# Autodesk Inventor assembly: X_CarriageFWDBearing_V2_1_Short
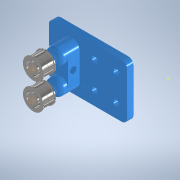
[picture p0: Inventor's stored thumbnail of the model, 180x180]
Saved by Autodesk Inventor 2022 (Build 260153000, 153)
## iProperties
Created: 2021-06-13
Part Number: X_CarriageFWDBearing_V2_1_Short
Document SubType Name: Assembly
Designer: Jorian Brusind
Author: Jorian Brusind
## Documents named in this file (6)
- C:\Users\Jorian Brusind\Documents\GitHub\HyperRail\Inventor Files\X_CarriageFWDBearing_V2_1_Short.iam
- C:\Users\Jorian Brusind\Documents\GitHub\HyperRail\Inventor Files\4mm_Roller_Spacer_simple.ipt
- C:\Users\Jorian Brusind\Documents\GitHub\HyperRail\Inventor Files\X_Carriage_Plate_Short.ipt
- C:\Users\Jorian Brusind\Documents\GitHub\HyperRail\Inventor Files\miniature-ball-bearings-metric-series-flanged-1.snapshot.1\F606ZZFlanged\F608 - 8 x 22 x 7.ipt
- C:\Users\Jorian Brusind\Documents\GitHub\PersonalProjects\HyperRail\Inventor Files\miniature-ball-bearings-metric-series-flanged-1.snapshot.1\F606ZZFlanged.ipt
- C:\Users\Jorian Brusind\Documents\GitHub\HyperRail\Inventor Files\Metric bolt\Bolt M5 45mm.ipt
## Components (8 placed, 4 different names)
1. X_Carriage_Plate_Short:1 — Mate:6, Mate:9, Angle:1, Mate:20
2. 4mm_Roller_Spacer_simple:1 — Mate:6, Mate:9, Angle:1, Mate:14, Mate:15, Mate:16, Mate:17, Mate:18, Mate:19
3. F608 - 8 x 22 x 7:4 — Mate:10, Mate:11
4. F608 - 8 x 22 x 7:5 — Mate:10, Mate:11, Mate:14, Mate:15
5. F608 - 8 x 22 x 7:6 — Mate:16
6. F608 - 8 x 22 x 7:7 — Mate:17
7. Bolt M5 45mm:1 — Mate:19, Mate:20, Flush:1
8. Bolt M5 45mm:2 — Mate:18, Flush:1
## Relationships (15: Mate 13, Angle 1, Flush 1)
- Mate:6: X_Carriage_Plate_Short:1 ↔ 4mm_Roller_Spacer_simple:1
- Mate:9 (-12.5 mm): X_Carriage_Plate_Short:1 ↔ 4mm_Roller_Spacer_simple:1
- Angle:1 (0 deg): X_Carriage_Plate_Short:1 ↔ 4mm_Roller_Spacer_simple:1
- Mate:10: F608 - 8 x 22 x 7:4 ↔ F608 - 8 x 22 x 7:5
- Mate:11: F608 - 8 x 22 x 7:4 ↔ F608 - 8 x 22 x 7:5
- [Mate]: F608 - 8 x 22 x 7:6 ↔ F608 - 8 x 22 x 7:7
- [Mate]: F608 - 8 x 22 x 7:6 ↔ F608 - 8 x 22 x 7:7
- Mate:14: 4mm_Roller_Spacer_simple:1 ↔ F608 - 8 x 22 x 7:5
- Mate:15: 4mm_Roller_Spacer_simple:1 ↔ F608 - 8 x 22 x 7:5
- Mate:16: 4mm_Roller_Spacer_simple:1 ↔ F608 - 8 x 22 x 7:6
- Mate:17: 4mm_Roller_Spacer_simple:1 ↔ F608 - 8 x 22 x 7:7
- Mate:18: 4mm_Roller_Spacer_simple:1 ↔ Bolt M5 45mm:2
- Mate:19: 4mm_Roller_Spacer_simple:1 ↔ Bolt M5 45mm:1
- Mate:20: X_Carriage_Plate_Short:1 ↔ Bolt M5 45mm:1
- Flush:1: Bolt M5 45mm:1 ↔ Bolt M5 45mm:2
## Named parameters: d100_d98 = 0 mm, d101_d99 = 0 mm
